# Autodesk Inventor assembly: Support
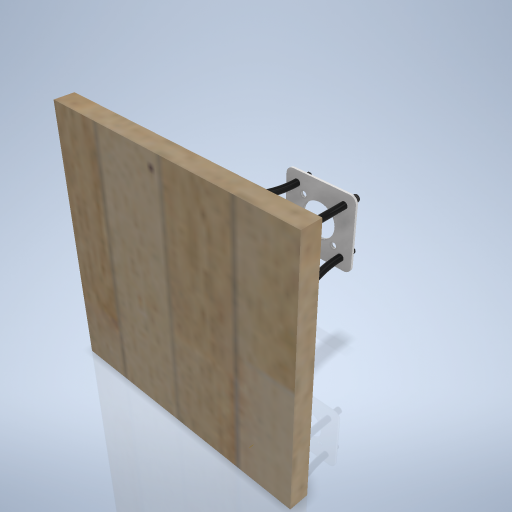
[picture p0: Inventor's stored thumbnail of the model, 512x512]
Saved by Autodesk Inventor 2024.2 (Build 282272000, 272)
## iProperties
Created: 2024-05-16
Part Number: Support
Document SubType Name: Assembly
Designer: Fabri
Author: Fabri
## Documents named in this file (4)
- C:\Users\Fabri\Documents\Inventor\Stirlingfan\Support.iam
- C:\Users\Fabri\Documents\Inventor\Stirlingfan\wooden support.ipt
- C:\Users\Fabri\Documents\Inventor\Stirlingfan\stand.ipt
- C:\Users\Fabri\Documents\Inventor\Stirlingfan\12.ipt
## Components (6 placed, 3 different names)
1. wooden support:1 — Passend:1, Passend:2, Passend:3, Passend:4, Fluchtend:1, Fluchtend:2
2. stand:3 — Passend:1, Winkel:1, Symmetrie:1, Einfügen:1
3. stand:4 — Passend:2, Winkel:2, Symmetrie:1, Symmetrie:3
4. stand:5 — Passend:4, Winkel:3, Symmetrie:2
5. stand:6 — Passend:3, Winkel:4, Symmetrie:2, Symmetrie:3
6. 12:1 — Einfügen:1
## Relationships (14: Mate 4, Angle 4, Symmetry 3, Flush 2, Insert 1)
- Passend:1 [Mate]: wooden support:1 ↔ stand:3
- Winkel:1 [Angle] (45 deg): stand:3
- Passend:2 [Mate]: wooden support:1 ↔ stand:4
- Winkel:2 [Angle] (-45 deg): stand:4
- Passend:3 [Mate]: wooden support:1 ↔ stand:6
- Passend:4 [Mate]: wooden support:1 ↔ stand:5
- Winkel:3 [Angle] (135 deg): stand:5
- Winkel:4 [Angle] (225 deg): stand:6
- Fluchtend:1 [Flush]: wooden support:1
- Symmetrie:1: stand:3 ↔ stand:4
- Fluchtend:2 [Flush]: wooden support:1
- Symmetrie:2: stand:5 ↔ stand:6
- Symmetrie:3: stand:4 ↔ stand:6
- Einfügen:1 [Insert] (-13 mm): stand:3 ↔ 12:1
